# Autodesk Inventor assembly: Złożenie całości
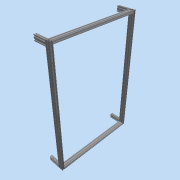
[picture p0: Inventor's stored thumbnail of the model, 180x180]
Saved by Autodesk Inventor 2018 (Build 220112000, 112)
## iProperties
Created: 2019-01-23
Part Number: Złożenie całości
Material: Ogólny
Document SubType Name: Assembly
Designer: Dawid
Author: Dawid
## Documents named in this file (4)
- E:\Frezarka_K2\INVENTOR\ZŁOŻENIA\Złożenie całości.iam
- E:\Frezarka_K2\INVENTOR\RAMA\Profil dolny długi.ipt
- E:\Frezarka_K2\INVENTOR\RAMA\Profil dolny krótki.ipt
- E:\Frezarka_K2\INVENTOR\RAMA\Profil dolny - noga.ipt
## Components (8 placed, 3 different names)
1. Profil dolny długi:1 — Zestawiający:1, Równoległy:1, Równoległy:2, Zestawiający:4, Równoległy:7, Zestawiający:7, Równoległy:13, Równoległy:14
2. Profil dolny krótki:1 — Zestawiający:1, Równoległy:1, Równoległy:2, Zestawiający:2, Równoległy:3, Równoległy:4
3. Profil dolny długi:2 — Zestawiający:2, Równoległy:3, Równoległy:4, Zestawiający:3, Równoległy:5, Równoległy:6, Zestawiający:5, Równoległy:9, Równoległy:10, Zestawiający:6, Równoległy:11, Równoległy:12
4. Profil dolny krótki:2 — Zestawiający:3, Równoległy:5, Równoległy:6, Równoległy:8
5. Profil dolny - noga:1 — Zestawiający:5, Równoległy:9, Równoległy:10
6. Profil dolny - noga:2 — Zestawiający:6, Równoległy:11, Równoległy:12
7. Profil dolny - noga:3 — Zestawiający:7, Równoległy:13, Równoległy:14
8. Profil dolny - noga:4 — Zestawiający:4, Równoległy:7, Równoległy:8
## Relationships (21: Flush 14, Mate 7)
- Zestawiający:1 [Mate]: Profil dolny długi:1 ↔ Profil dolny krótki:1
- Równoległy:1 [Flush]: Profil dolny długi:1 ↔ Profil dolny krótki:1
- Równoległy:2 [Flush]: Profil dolny długi:1 ↔ Profil dolny krótki:1
- Zestawiający:2 [Mate]: Profil dolny krótki:1 ↔ Profil dolny długi:2
- Równoległy:3 [Flush]: Profil dolny krótki:1 ↔ Profil dolny długi:2
- Równoległy:4 [Flush]: Profil dolny krótki:1 ↔ Profil dolny długi:2
- Zestawiający:3 [Mate]: Profil dolny długi:2 ↔ Profil dolny krótki:2
- Równoległy:5 [Flush]: Profil dolny długi:2 ↔ Profil dolny krótki:2
- Równoległy:6 [Flush]: Profil dolny długi:2 ↔ Profil dolny krótki:2
- Zestawiający:4 [Mate]: Profil dolny długi:1 ↔ Profil dolny - noga:4
- Równoległy:7 [Flush]: Profil dolny długi:1 ↔ Profil dolny - noga:4
- Równoległy:8 [Flush]: Profil dolny krótki:2 ↔ Profil dolny - noga:4
- Zestawiający:5 [Mate]: Profil dolny długi:2 ↔ Profil dolny - noga:1
- Równoległy:9 [Flush]: Profil dolny długi:2 ↔ Profil dolny - noga:1
- Równoległy:10 [Flush]: Profil dolny długi:2 ↔ Profil dolny - noga:1
- Zestawiający:6 [Mate]: Profil dolny długi:2 ↔ Profil dolny - noga:2
- Równoległy:11 [Flush]: Profil dolny długi:2 ↔ Profil dolny - noga:2
- Równoległy:12 [Flush]: Profil dolny długi:2 ↔ Profil dolny - noga:2
- Zestawiający:7 [Mate]: Profil dolny długi:1 ↔ Profil dolny - noga:3
- Równoległy:13 [Flush]: Profil dolny długi:1 ↔ Profil dolny - noga:3
- Równoległy:14 [Flush]: Profil dolny długi:1 ↔ Profil dolny - noga:3
